# Autodesk Inventor assembly: adjustable_arm
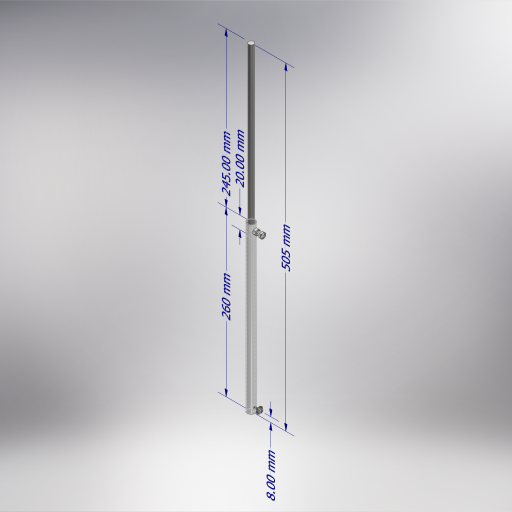
[picture p0: Inventor's stored thumbnail of the model, 512x512]
Saved by Autodesk Inventor 2023 (Build 270158030, 158C)
## iProperties
Created: 2022-04-27
Part Number: adjustable_arm
Document SubType Name: Assembly
Designer: Norbert Ligas
arm_min_length: 280,000 mm
arm_max_length: 505,000 mm
max_extrusion: 245,000 mm
min_extrusion: 20,000 mm
hinge_insertion: 15,000 mm
connection_length: 20,000 mm
bar_length: 265,000
pipe_length: 260,000 mm
bar_diameter: 8,000 mm
Author: Norbert Ligas
## Documents named in this file (7)
- C:\Users\norbe\Repozytoria\NormalMapScanner\3D_modeling\construction\parts\adjustable_arm.iam
- C:\Users\norbe\Repozytoria\NormalMapScanner\3D_modeling\construction\parts\pipe_300mm.ipt
- C:\Users\norbe\Repozytoria\NormalMapScanner\3D_modeling\construction\parts\bar_285mm.ipt
- C:\Users\norbe\OneDrive\Dokumenty\Inventor\Content Center Files\R2023\en-US\ISO 4032(2)\ISO 4032 - M5 - ISO.ipt
- C:\Users\norbe\OneDrive\Dokumenty\Inventor\Content Center Files\R2023\en-US\ISO 4017(1)\ISO 4017 - M5 x 16 - ISO.ipt
- C:\Users\norbe\OneDrive\Dokumenty\Inventor\Content Center Files\R2023\en-US\ISO 7045  Z\ISO 7045 - M3,5 x 14_ - 4.8 - Z - ISO.ipt
- C:\Users\norbe\OneDrive\Dokumenty\Inventor\Content Center Files\R2023\en-US\ISO 7090\ISO 7090 - 5 - 140 HV(1).ipt
## Components (6 placed, 6 different names)
1. pipe_300mm:1 — Cylindrical:1, Mate:1, Mate:2, Mate:3, Tangent:1, Mate:4, Mate:5, Tangent:2
2. bar_285mm:1 — Cylindrical:1
3. ISO 4032 M5:1 — Tangent:1, Mate:4, Insert:1
4. ISO 4017 M5 x 16:1 — Insert:1
5. ISO 7045 Z M3,5 x 14 - 4.8 - Z:1 — Mate:5, Mate:6, Mate:7
6. ISO 7090 5 - 140 HV:1 — Mate:6, Mate:7, Tangent:2
## Relationships (11: Mate 7, Tangent 2, CylindricalJoint 1, Insert 1)
- Cylindrical:1: pipe_300mm:1 ↔ bar_285mm:1
- Mate:1: pipe_300mm:1
- Mate:2: pipe_300mm:1
- Mate:3: pipe_300mm:1
- Tangent:1: pipe_300mm:1 ↔ ISO 4032 M5:1
- Mate:4: pipe_300mm:1 ↔ ISO 4032 M5:1
- Insert:1 (5 mm): ISO 4032 M5:1 ↔ ISO 4017 M5 x 16:1
- Mate:5: pipe_300mm:1 ↔ ISO 7045 Z M3,5 x 14 - 4.8 - Z:1
- Mate:6: ISO 7045 Z M3,5 x 14 - 4.8 - Z:1 ↔ ISO 7090 5 - 140 HV:1
- Mate:7: ISO 7045 Z M3,5 x 14 - 4.8 - Z:1 ↔ ISO 7090 5 - 140 HV:1
- Tangent:2 (7 mm): pipe_300mm:1 ↔ ISO 7090 5 - 140 HV:1
## Named parameters: arm_min_length = 280 mm, arm_max_length = 505 mm, max_extrusion = 245 mm, min_extrusion = 20 mm, hinge_insertion = 15 mm, connection_length = 20 mm, bar_length = 265 mm, pipe_length = 260 mm, bar_diameter = 8 mm, stand_diameter = 800 mm, hinge_insertion_1 = 15 mm, connection_length_1 = 20 mm, box_diameter = 200 mm, hinge_arm_length = 25 mm, margin_for_connection = 10 mm
